# Autodesk Inventor assembly: Structure
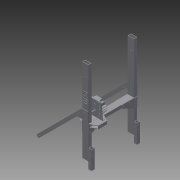
[picture p0: Inventor's stored thumbnail of the model, 180x180]
Saved by Autodesk Inventor 2013 (Build 170138000, 138)
## iProperties
Created: 2014-01-22
Part Number: Structure
Document SubType Name: Assembly
Designer: Jarod
Author: Jarod
## Documents named in this file (9)
- E:\Robotics\FRC\2014\CAD\Robot\Catapult\Structure.iam
- E:\Robotics\FRC\2014\CAD\Robot\Catapult\Structure\SuperSuperStructure.ipt
- E:\Robotics\FRC\2014\CAD\Robot\Catapult\Structure\MotorSupport.ipt
- E:\Robotics\FRC\2014\CAD\Robot\Catapult\Structure\SideGusset.ipt
- E:\Robotics\FRC\2014\CAD\Robot\Catapult\Structure\SideSupport.ipt
- E:\Robotics\FRC\2014\CAD\Robot\Catapult\Structure\CatapultGussetPlate.ipt
- E:\Robotics\FRC\2014\CAD\Robot\Catapult\Structure\CatapultMotorSupport.ipt
- E:\Robotics\FRC\2014\CAD\Robot\Catapult\Structure\SuperStructureSupport.ipt
- C:\Users\Jarod\Documents\Inventor\Toughbox-mini.iam
## Components (16 placed, 8 different names)
1. SuperSuperStructure:1 — Mate:1, Flush:1, Flush:2, Mate:2, Flush:3, Mate:3, Mate:6, Mate:7, Flush:5, Mate:24, Mate:25, Flush:15, Mate:27, Flush:19
2. SuperSuperStructure:2 — Mate:1, Flush:1, Flush:2, Mate:4, Flush:4, Mate:5, Mate:8, Mate:9, Flush:6, Mate:26, Flush:17
3. MotorSupport:1 — Mate:18, Mate:19, Flush:11, Flush:13, Mate:22
4. MotorSupport:2 — Mate:20, Mate:21, Flush:12, Flush:14
5. SideGusset:1 — Mate:6, Mate:7, Flush:5, Flush:16
6. SideGusset:2 — Mate:8, Mate:9, Flush:6, Flush:18
7. SideSupport:1 — Mate:25, Flush:15, Flush:16
8. SideSupport:2 — Mate:26, Flush:17, Flush:18
9. CatapultGussetPlate:1 — Mate:16, Flush:10, Mate:17
10. CatapultGussetPlate:2 — Mate:14, Flush:9, Mate:15, Mate:20, Mate:21, Mate:27
11. CatapultGussetPlate:3 — Mate:12, Flush:8, Mate:13
12. CatapultGussetPlate:4 — Mate:10, Flush:7, Mate:11, Mate:18, Mate:19
13. CatapultMotorSupport:1 — Mate:10, Flush:7, Mate:11, Mate:12, Flush:8, Mate:13, Mate:14, Flush:9, Mate:15, Mate:16, Flush:10, Mate:17, Flush:11, Flush:12, Mate:23, Mate:24, Flush:19
14. SuperStructureSupport:1 — Mate:2, Flush:3, Mate:3
15. SuperStructureSupport:2 — Mate:4, Flush:4, Mate:5
16. Toughbox-mini:1 [sub-assembly] — Flush:13, Mate:22, Mate:23, Flush:14
## Relationships (46: Mate 27, Flush 19)
- Mate:1 (349.25 mm): SuperSuperStructure:1 ↔ SuperSuperStructure:2
- Flush:1: SuperSuperStructure:1 ↔ SuperSuperStructure:2
- Flush:2: SuperSuperStructure:1 ↔ SuperSuperStructure:2
- Mate:2: SuperSuperStructure:1 ↔ SuperStructureSupport:1
- Flush:3: SuperSuperStructure:1 ↔ SuperStructureSupport:1
- Mate:3: SuperSuperStructure:1 ↔ SuperStructureSupport:1
- Mate:4: SuperSuperStructure:2 ↔ SuperStructureSupport:2
- Flush:4: SuperSuperStructure:2 ↔ SuperStructureSupport:2
- Mate:5: SuperSuperStructure:2 ↔ SuperStructureSupport:2
- Mate:6: SuperSuperStructure:1 ↔ SideGusset:1
- Mate:7: SuperSuperStructure:1 ↔ SideGusset:1
- Flush:5: SuperSuperStructure:1 ↔ SideGusset:1
- Mate:8: SuperSuperStructure:2 ↔ SideGusset:2
- Mate:9: SuperSuperStructure:2 ↔ SideGusset:2
- Flush:6: SuperSuperStructure:2 ↔ SideGusset:2
- Mate:10: CatapultGussetPlate:4 ↔ CatapultMotorSupport:1
- Flush:7: CatapultGussetPlate:4 ↔ CatapultMotorSupport:1
- Mate:11: CatapultGussetPlate:4 ↔ CatapultMotorSupport:1
- Mate:12: CatapultGussetPlate:3 ↔ CatapultMotorSupport:1
- Flush:8: CatapultGussetPlate:3 ↔ CatapultMotorSupport:1
- Mate:13: CatapultGussetPlate:3 ↔ CatapultMotorSupport:1
- Mate:14: CatapultGussetPlate:2 ↔ CatapultMotorSupport:1
- Flush:9: CatapultGussetPlate:2 ↔ CatapultMotorSupport:1
- Mate:15: CatapultGussetPlate:2 ↔ CatapultMotorSupport:1
- Mate:16: CatapultGussetPlate:1 ↔ CatapultMotorSupport:1
- Flush:10: CatapultGussetPlate:1 ↔ CatapultMotorSupport:1
- Mate:17: CatapultGussetPlate:1 ↔ CatapultMotorSupport:1
- Mate:18: MotorSupport:1 ↔ CatapultGussetPlate:4
- Mate:19: MotorSupport:1 ↔ CatapultGussetPlate:4
- Flush:11: MotorSupport:1 ↔ CatapultMotorSupport:1
- Mate:20: MotorSupport:2 ↔ CatapultGussetPlate:2
- Mate:21: MotorSupport:2 ↔ CatapultGussetPlate:2
- Flush:12: MotorSupport:2 ↔ CatapultMotorSupport:1
- Flush:13 (15.875 mm): MotorSupport:1 ↔ Toughbox-mini:1
- Mate:22 (3.175 mm): MotorSupport:1 ↔ Toughbox-mini:1
- Mate:23: CatapultMotorSupport:1 ↔ Toughbox-mini:1
- Flush:14 (15.875 mm): MotorSupport:2 ↔ Toughbox-mini:1
- Mate:24: SuperSuperStructure:1 ↔ CatapultMotorSupport:1
- Mate:25: SuperSuperStructure:1 ↔ SideSupport:1
- Flush:15: SuperSuperStructure:1 ↔ SideSupport:1
- Flush:16: SideGusset:1 ↔ SideSupport:1
- Mate:26: SuperSuperStructure:2 ↔ SideSupport:2
- Flush:17: SuperSuperStructure:2 ↔ SideSupport:2
- Flush:18: SideGusset:2 ↔ SideSupport:2
- Mate:27: SuperSuperStructure:1 ↔ CatapultGussetPlate:2
- Flush:19 (419.1 mm): SuperSuperStructure:1 ↔ CatapultMotorSupport:1
